# Autodesk Inventor assembly: Assembly1
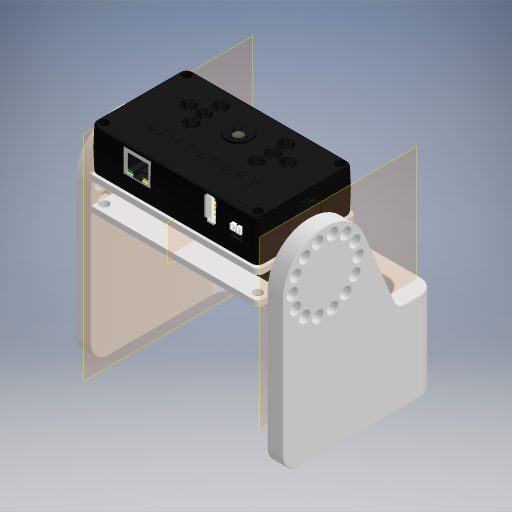
[picture p0: Inventor's stored thumbnail of the model, 512x512]
Saved by Autodesk Inventor 2024.2 (Build 282272000, 272)
## iProperties
Created: 2024-02-01
Part Number: Assembly1
Document SubType Name: Assembly
Designer: rohan
Author: rohan
## Documents named in this file (5)
- C:\Users\rohan\OneDrive - Hillsborough County Public Schools\Robotics\FIRST-Robotics-Competition\Crescendo\Minotaur-Crescendo-Robot\Structure\New folder\Assembly1.iam
- C:\Users\rohan\OneDrive - Hillsborough County Public Schools\Robotics\FIRST-Robotics-Competition\Crescendo\Minotaur-Crescendo-Robot\Electronics\Limelight-2.ipt
- C:\Users\rohan\OneDrive - Hillsborough County Public Schools\Robotics\FIRST-Robotics-Competition\Crescendo\Minotaur-Crescendo-Robot\Structure\New folder\Limelight.ipt
- C:\Users\rohan\OneDrive - Hillsborough County Public Schools\Robotics\FIRST-Robotics-Competition\Crescendo\Minotaur-Crescendo-Robot\Structure\New folder\Part4.ipt
- C:\Users\rohan\OneDrive - Hillsborough County Public Schools\Robotics\FIRST-Robotics-Competition\Crescendo\Minotaur-Crescendo-Robot\Structure\New folder\Part6.ipt
## Components (6 placed, 4 different names)
1. Limelight-2:1 — Mate:1, Insert:1, Insert:2
2. Limelight:1 — Mate:1, Insert:1, Insert:2, Mate:2, Mate:3, Mate:5, Mate:6, Symmetry:1
3. Part4:3 — Mate:3, Mate:4, Flush:1, Symmetry:2
4. Part4:4 — Mate:2, Flush:1, Symmetry:2
5. Limelight:2 — Mate:4, Mate:5, Mate:6, Symmetry:1
6. Part6:1
## Relationships (11: Mate 6, Insert 2, Symmetry 2, Flush 1)
- Mate:1: Limelight-2:1 ↔ Limelight:1
- Insert:1: Limelight-2:1 ↔ Limelight:1
- Insert:2: Limelight-2:1 ↔ Limelight:1
- Mate:2: Limelight:1 ↔ Part4:4
- Mate:3: Limelight:1 ↔ Part4:3
- Mate:4: Part4:3 ↔ Limelight:2
- Mate:5: Limelight:1 ↔ Limelight:2
- Mate:6: Limelight:1 ↔ Limelight:2
- Symmetry:1: Limelight:1 ↔ Limelight:2
- Flush:1: Part4:3 ↔ Part4:4
- Symmetry:2: Part4:3 ↔ Part4:4
